# Autodesk Inventor assembly: hcsr04
Saved by Autodesk Inventor 2021 (Build 250183000, 183)
## iProperties
Company: Unknown
Created: 2018-10-29
Part Number: hcsr04
Description: Unknown
Document SubType Name: Assembly
Designer: User
Sending System: DEX
Preprocessor: ST-DEVELOPER v16.7
Title: HC-SR04
Author: Unknown
## Documents named in this file (9)
- D:\SynologyDrive\tcodev\tco-cad\common\hcsr04\hcsr04.iam
- D:\SynologyDrive\tcodev\tco-cad\common\hcsr04\Board.ipt
- D:\SynologyDrive\tcodev\tco-cad\common\kicad_packages_3d\SOIC-16_3.9x9.9mm_P1.27mm.ipt
- D:\SynologyDrive\tcodev\tco-cad\common\kicad_packages_3d\SOIC-14_3.9x8.7mm_P1.27mm.ipt
- D:\SynologyDrive\tcodev\tco-cad\common\kicad_packages_3d\C_0603_1608Metric.ipt
- D:\SynologyDrive\tcodev\tco-cad\common\kicad_packages_3d\R_0603_1608Metric.ipt
- D:\SynologyDrive\tcodev\tco-cad\common\kicad_packages_3d\PinHeader_1x04_P2.54mm_Horizontal.ipt
- D:\SynologyDrive\tcodev\tco-cad\common\kicad_packages_3d\Crystal_HC49-4H_Vertical.ipt
- D:\SynologyDrive\tcodev\tco-cad\common\hcsr04\Transducer.iam
## Components (20 placed, 8 different names)
1. Board — Mate:4, Angle:3, Mate:5, Mate:6, Angle:4, Angle:5, Mate:7, Mate:8, Mate:9, Mate:10, Mate:11, Mate:12, Mate:13, Mate:14, Mate:15, Rigid:1, Rigid:2, Mate:16, Mate:17, Rigid:3, Rotational:1
2. Crystal_HC49-4H_Vertical:1 — Rigid:2
3. SOIC-16_3.9x9.9mm_P1.27mm:3 — Mate:4, Angle:3
4. SOIC-14_3.9x8.7mm_P1.27mm:1 — Mate:5, Angle:4
5. SOIC-14_3.9x8.7mm_P1.27mm:2 — Mate:6, Angle:5
6. C_0603_1608Metric:4 — Mate:9, Flush:3, Flush:8, Flush:13
7. C_0603_1608Metric:5 — Mate:10, Flush:3, Flush:4, Flush:8, Flush:9
8. C_0603_1608Metric:6 — Mate:11, Flush:5, Flush:6, Flush:10, Flush:11
9. R_0603_1608Metric:4 — Mate:12, Flush:4, Flush:5, Flush:9, Flush:10
10. R_0603_1608Metric:5 — Mate:13, Flush:6, Flush:7, Flush:11, Flush:12
11. R_0603_1608Metric:6 — Mate:14, Flush:7, Flush:12
12. PinHeader_1x04_P2.54mm_Horizontal:1 — Mate:15, Rigid:1
13. Transducer:1 [sub-assembly] — Mate:17, Rigid:3
14. Transducer:2 [sub-assembly] — Mate:16, Rotational:1
15. R_0603_1608Metric:1 — Mate:8, Flush:2, Flush:13
16. R_0603_1608Metric:2
17. R_0603_1608Metric:3
18. C_0603_1608Metric:1 — Mate:7, Flush:2
19. C_0603_1608Metric:2
20. C_0603_1608Metric:3
## Component patterns: (3 elements, first: R_0603_1608Metric:1), (3 elements, first: C_0603_1608Metric:1)
## Relationships (33: Mate 14, Flush 12, Angle 3, WeldJoint 3, RevoluteJoint 1)
- Mate:4: Board ↔ SOIC-16_3.9x9.9mm_P1.27mm:3
- Angle:3 (0 deg): Board ↔ SOIC-16_3.9x9.9mm_P1.27mm:3
- Mate:5: Board ↔ SOIC-14_3.9x8.7mm_P1.27mm:1
- Mate:6: Board ↔ SOIC-14_3.9x8.7mm_P1.27mm:2
- Angle:4 (0 deg): Board ↔ SOIC-14_3.9x8.7mm_P1.27mm:1
- Angle:5 (0 deg): Board ↔ SOIC-14_3.9x8.7mm_P1.27mm:2
- Mate:7: Board ↔ C_0603_1608Metric:1
- Mate:8: Board ↔ R_0603_1608Metric:1
- Flush:2: R_0603_1608Metric:1 ↔ C_0603_1608Metric:1
- Mate:9: Board ↔ C_0603_1608Metric:4
- Mate:10: Board ↔ C_0603_1608Metric:5
- Mate:11: Board ↔ C_0603_1608Metric:6
- Mate:12: Board ↔ R_0603_1608Metric:4
- Mate:13: Board ↔ R_0603_1608Metric:5
- Mate:14: Board ↔ R_0603_1608Metric:6
- Flush:3: C_0603_1608Metric:4 ↔ C_0603_1608Metric:5
- Flush:4: C_0603_1608Metric:5 ↔ R_0603_1608Metric:4
- Flush:5: C_0603_1608Metric:6 ↔ R_0603_1608Metric:4
- Flush:6: C_0603_1608Metric:6 ↔ R_0603_1608Metric:5
- Flush:7: R_0603_1608Metric:5 ↔ R_0603_1608Metric:6
- Flush:8 (2.15 mm): C_0603_1608Metric:4 ↔ C_0603_1608Metric:5
- Flush:9 (2.15 mm): C_0603_1608Metric:5 ↔ R_0603_1608Metric:4
- Flush:10 (2.15 mm): C_0603_1608Metric:6 ↔ R_0603_1608Metric:4
- Flush:11 (2.15 mm): C_0603_1608Metric:6 ↔ R_0603_1608Metric:5
- Flush:12 (2.15 mm): R_0603_1608Metric:5 ↔ R_0603_1608Metric:6
- Mate:15: Board ↔ PinHeader_1x04_P2.54mm_Horizontal:1
- Rigid:1 [WeldJoint] (-3 mm): Board ↔ PinHeader_1x04_P2.54mm_Horizontal:1
- Rigid:2 [WeldJoint] (-3 mm): Board ↔ Crystal_HC49-4H_Vertical:1
- Mate:16: Board ↔ Transducer:2
- Mate:17: Board ↔ Transducer:1
- Rigid:3 [WeldJoint] (-3 mm): Board ↔ Transducer:1
- Rotational:1 [RevoluteJoint] (-3 mm): Board ↔ Transducer:2
- Flush:13: C_0603_1608Metric:4 ↔ R_0603_1608Metric:1
